# Autodesk Inventor assembly: McCrea_car_walle
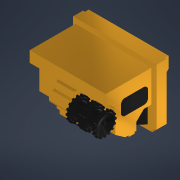
[picture p0: Inventor's stored thumbnail of the model, 180x180]
Saved by Autodesk Inventor 2022 (Build 260153000, 153)
## iProperties
Created: 2022-02-07
Part Number: McCrea_car_walle
Document SubType Name: Assembly
Designer: MatusBarany
Author: MatusBarany
## Documents named in this file (4)
- C:\Users\MatusBarany\Documents\Inventor\wall-e\assembly\McCrea_car_walle.iam
- C:\Users\MatusBarany\Documents\Inventor\wall-e\matus\electronic truck\McCrea_front_walle.ipt
- C:\Users\MatusBarany\Documents\Inventor\wall-e\matus\electronic truck\McCrea_front_wheel_walle.ipt
- C:\Users\MatusBarany\Documents\Inventor\wall-e\matus\electronic truck\McCrea_roof_walle.ipt
## Components (4 placed, 3 different names)
1. McCrea_front_walle:1 — Mate:1, Mate:2, Flush:1, Rigid:1
2. McCrea_front_wheel_walle:1 — Rigid:2
3. McCrea_roof_walle:1 — Mate:1, Mate:2, Flush:1
4. McCrea_front_wheel_walle:2 — Rigid:1, Rigid:2
## Relationships (5: Mate 2, WeldJoint 2, Flush 1)
- Mate:1: McCrea_front_walle:1 ↔ McCrea_roof_walle:1
- Mate:2: McCrea_front_walle:1 ↔ McCrea_roof_walle:1
- Flush:1: McCrea_front_walle:1 ↔ McCrea_roof_walle:1
- Rigid:1 [WeldJoint]: McCrea_front_walle:1 ↔ McCrea_front_wheel_walle:2
- Rigid:2 [WeldJoint]: McCrea_front_wheel_walle:1 ↔ McCrea_front_wheel_walle:2
